# Autodesk Inventor assembly: Frame
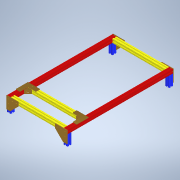
[picture p0: Inventor's stored thumbnail of the model, 180x180]
Saved by Autodesk Inventor 2022.3 (Build 263350000, 350)
## iProperties
Created: 2022-03-31
Part Number: Frame
Document SubType Name: Assembly
Designer: Robert Nies
Author: Robert Nies
## Documents named in this file (7)
- C:\Users\rober\PycharmProjects\CNCRouter\Master Assembly\Frame\Frame.iam
- C:\Users\rober\PycharmProjects\CNCRouter\Master Assembly\Frame\Frame Short.ipt
- C:\Users\rober\PycharmProjects\CNCRouter\Master Assembly\Frame\Leg.ipt
- C:\Users\rober\PycharmProjects\CNCRouter\Stock Parts\Brackets\90 Deg 5 Hole Bracket.ipt
- C:\Users\rober\PycharmProjects\CNCRouter\Stock Parts\Brackets\Inside Corner Bracket.ipt
- C:\Users\rober\PycharmProjects\CNCRouter\Stock Parts\Brackets\L Bracket.ipt
- C:\Users\rober\PycharmProjects\CNCRouter\Master Assembly\Frame\Frame Long _ ALT.ipt
## Components (17 placed, 6 different names)
1. Frame Short:2 — Flush:15, Flush:16, Angle:4, Tangent:2
2. Frame Short:1 — Angle:1, Tangent:1, Mate:1, Angle:2, Flush:2, Mate:7, Flush:11, Mate:10, Angle:3
3. Frame Long _ ALT:2 — Flush:1, Mate:2, Flush:2, Flush:6, Mate:3, Mate:4, Flush:20, Flush:22, Mate:15, Flush:23
4. Frame Long _ ALT:1 — Flush:11, Mate:11, Flush:12, Mate:12, Flush:14, Flush:15, Mate:13, Flush:18, Flush:24, Mate:17, Flush:25, Mate:18, Mate:19, Mate:21, Flush:28
5. Frame Short:3 — Flush:7, Flush:8, Mate:7, Flush:10, Mate:9, Flush:26, Mate:20
6. Leg:8 — Mate:14, Mate:15, Flush:23
7. Leg:7 — Mate:16, Flush:24, Mate:17
8. Leg:2 — Mate:21, Mate:23, Flush:28
9. Leg:1 — Mate:4, Mate:5, Mate:6
10. Inside Corner Bracket:1 — Mate:19, Mate:20, Flush:27
11. Inside Corner Bracket:2 — Flush:3, Flush:4, Mate:9
12. L Bracket:1 — Flush:9, Mate:8, Flush:10
13. L Bracket:2 — Flush:25, Mate:18, Flush:26
14. 90 Deg 5 Hole Bracket:3 — Flush:5, Flush:6, Mate:3, Mate:5, Flush:9
15. 90 Deg 5 Hole Bracket:6 — Flush:17, Flush:18, Flush:19, Mate:16
16. 90 Deg 5 Hole Bracket:7 — Flush:20, Flush:21, Flush:22, Mate:14
17. 90 Deg 5 Hole Bracket:1 — Mate:12, Flush:13, Flush:14, Mate:23
## Relationships (56: Flush 28, Mate 22, Angle 4, Tangent 2)
- Angle:1 (0 deg): Frame Short:1
- Tangent:1: Frame Short:1
- Flush:1: Frame Long _ ALT:2
- Mate:1: Frame Short:1
- Angle:2 (0 deg): Frame Short:1
- Mate:2: Frame Long _ ALT:2
- Flush:2: Frame Short:1 ↔ Frame Long _ ALT:2
- Flush:3: Inside Corner Bracket:2
- Flush:4: Inside Corner Bracket:2
- Flush:5: 90 Deg 5 Hole Bracket:3
- Flush:6: Frame Long _ ALT:2 ↔ 90 Deg 5 Hole Bracket:3
- Mate:3: Frame Long _ ALT:2 ↔ 90 Deg 5 Hole Bracket:3
- Mate:4: Frame Long _ ALT:2 ↔ Leg:1
- Mate:5: Leg:1 ↔ 90 Deg 5 Hole Bracket:3
- Mate:6: Leg:1
- Flush:7: Frame Short:3
- Flush:8: Frame Short:3
- Mate:7 (127 mm): Frame Short:1 ↔ Frame Short:3
- Flush:9: L Bracket:1 ↔ 90 Deg 5 Hole Bracket:3
- Mate:8: L Bracket:1
- Flush:10: Frame Short:3 ↔ L Bracket:1
- Mate:9: Frame Short:3 ↔ Inside Corner Bracket:2
- Flush:11: Frame Short:1 ↔ Frame Long _ ALT:1
- Mate:10: Frame Short:1
- Angle:3 (0 deg): Frame Short:1
- Mate:11: Frame Long _ ALT:1
- Flush:12: Frame Long _ ALT:1
- Mate:12: Frame Long _ ALT:1 ↔ 90 Deg 5 Hole Bracket:1
- Flush:13: 90 Deg 5 Hole Bracket:1
- Flush:14: Frame Long _ ALT:1 ↔ 90 Deg 5 Hole Bracket:1
- Flush:15: Frame Short:2 ↔ Frame Long _ ALT:1
- Flush:16: Frame Short:2
- Angle:4 (0 deg): Frame Short:2
- Tangent:2: Frame Short:2
- Mate:13: Frame Long _ ALT:1
- Flush:17: 90 Deg 5 Hole Bracket:6
- Flush:18: Frame Long _ ALT:1 ↔ 90 Deg 5 Hole Bracket:6
- Flush:19: 90 Deg 5 Hole Bracket:6
- Flush:20: Frame Long _ ALT:2 ↔ 90 Deg 5 Hole Bracket:7
- Flush:21: 90 Deg 5 Hole Bracket:7
- Flush:22: Frame Long _ ALT:2 ↔ 90 Deg 5 Hole Bracket:7
- Mate:14: Leg:8 ↔ 90 Deg 5 Hole Bracket:7
- Mate:15: Frame Long _ ALT:2 ↔ Leg:8
- Flush:23: Frame Long _ ALT:2 ↔ Leg:8
- Mate:16: Leg:7 ↔ 90 Deg 5 Hole Bracket:6
- Flush:24: Frame Long _ ALT:1 ↔ Leg:7
- Mate:17: Frame Long _ ALT:1 ↔ Leg:7
- Flush:25: Frame Long _ ALT:1 ↔ L Bracket:2
- Mate:18: Frame Long _ ALT:1 ↔ L Bracket:2
- Flush:26: Frame Short:3 ↔ L Bracket:2
- Mate:19: Frame Long _ ALT:1 ↔ Inside Corner Bracket:1
- Mate:20: Frame Short:3 ↔ Inside Corner Bracket:1
- Flush:27: Inside Corner Bracket:1
- Mate:21: Frame Long _ ALT:1 ↔ Leg:2
- Mate:23: Leg:2 ↔ 90 Deg 5 Hole Bracket:1
- Flush:28: Frame Long _ ALT:1 ↔ Leg:2
